# Autodesk Inventor assembly: Controlpanel
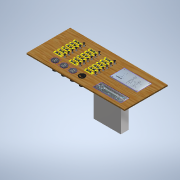
[picture p0: Inventor's stored thumbnail of the model, 180x180]
Saved by Autodesk Inventor 2021 (Build 250183000, 183)
## iProperties
Created: 2020-05-18
Part Number: Controlpanel
Document SubType Name: Assembly
Designer: Johansson
Author: Johansson
## Documents named in this file (10)
- C:\Users\oskar\Dropbox\Dokument\Projekt\Elita\Electrical system\Highside-Powerdistribution\hardware\control-panel\Controlpanel.iam
- C:\Users\oskar\Dropbox\Dokument\Projekt\Elita\Electrical system\Highside-Powerdistribution\hardware\control-panel\wooden-panel.ipt
- C:\Users\oskar\Dropbox\Dokument\Projekt\Elita\Electrical system\Highside-Powerdistribution\hardware\control-panel\label.ipt
- C:\Users\oskar\Dropbox\Dokument\Inventor\Content Center Files\R2019\en-US\CNS 9671\CNS 9671 - M2,3 x 5.ipt
- C:\Users\oskar\Dropbox\Dokument\Projekt\Elita\Electrical system\Highside-Powerdistribution\hardware\control-panel\stereo.ipt
- C:\Users\oskar\Dropbox\Dokument\Projekt\Elita\Electrical system\Highside-Powerdistribution\hardware\control-panel\usb_outlet.ipt
- C:\Users\oskar\Dropbox\Dokument\Projekt\Elita\Electrical system\Highside-Powerdistribution\hardware\control-panel\12v_outlet.ipt
- C:\Users\oskar\Dropbox\Dokument\Projekt\Elita\Electrical system\Highside-Powerdistribution\hardware\control-panel\dragswitch.ipt
- C:\Users\oskar\Dropbox\Dokument\Projekt\Elita\Electrical system\Highside-Powerdistribution\hardware\control-panel\infosign.ipt
- C:\Users\oskar\Dropbox\Dokument\Projekt\Elita\Electrical system\Highside-Powerdistribution\hardware\control-panel\parameters.xlsx
## Components (83 placed, 8 different names)
1. wooden-panel:1 — Mate:2, Mate:3, Mate:4, Mate:5, Mate:6, Mate:7, Mate:8, Mate:9, Mate:10, Mate:11, Mate:12
2. stereo:1 — Mate:3, Mate:4, Mate:5
3. 12v_outlet:1 — Mate:8, Mate:9
4. infosign:1 — Mate:12, Insert:5, Insert:6, Insert:7, Insert:8
5. CNS 9671 M2,3 x 5:45 — Insert:5
6. CNS 9671 M2,3 x 5:46 — Insert:6
7. CNS 9671 M2,3 x 5:47 — Insert:7
8. CNS 9671 M2,3 x 5:48 — Insert:8
9. label:5 — Mate:2, Insert:3, Insert:4
10. CNS 9671 M2,3 x 5:9 — Insert:3
11. CNS 9671 M2,3 x 5:10 — Insert:4
12. label:6
13. CNS 9671 M2,3 x 5:11
14. CNS 9671 M2,3 x 5:12
15. label:7
16. CNS 9671 M2,3 x 5:13
17. CNS 9671 M2,3 x 5:14
18. label:8
19. CNS 9671 M2,3 x 5:15
20. CNS 9671 M2,3 x 5:16
21. label:9
22. CNS 9671 M2,3 x 5:17
23. CNS 9671 M2,3 x 5:18
24. label:10
25. CNS 9671 M2,3 x 5:19
26. CNS 9671 M2,3 x 5:20
27. label:11
28. CNS 9671 M2,3 x 5:21
29. CNS 9671 M2,3 x 5:22
30. label:12
31. CNS 9671 M2,3 x 5:23
32. CNS 9671 M2,3 x 5:24
33. label:13
34. CNS 9671 M2,3 x 5:25
35. CNS 9671 M2,3 x 5:26
36. label:14
37. CNS 9671 M2,3 x 5:27
38. CNS 9671 M2,3 x 5:28
39. label:15
40. CNS 9671 M2,3 x 5:29
41. CNS 9671 M2,3 x 5:30
42. label:16
43. CNS 9671 M2,3 x 5:31
44. CNS 9671 M2,3 x 5:32
45. label:17
46. CNS 9671 M2,3 x 5:33
47. CNS 9671 M2,3 x 5:34
48. label:18
49. CNS 9671 M2,3 x 5:35
50. CNS 9671 M2,3 x 5:36
51. label:19
52. CNS 9671 M2,3 x 5:37
53. CNS 9671 M2,3 x 5:38
54. label:20
55. CNS 9671 M2,3 x 5:39
56. CNS 9671 M2,3 x 5:40
57. label:21
58. CNS 9671 M2,3 x 5:41
59. CNS 9671 M2,3 x 5:42
60. label:22
61. CNS 9671 M2,3 x 5:43
62. CNS 9671 M2,3 x 5:44
63. usb_outlet:1 — Mate:6, Mate:7
64. usb_outlet:2
65. usb_outlet:3
66. dragswitch:1 — Mate:10, Mate:11
67. dragswitch:2
68. dragswitch:3
69. dragswitch:4
70. dragswitch:5
71. dragswitch:6
72. dragswitch:7
73. dragswitch:8
74. dragswitch:9
75. dragswitch:10
76. dragswitch:11
77. dragswitch:12
78. dragswitch:13
79. dragswitch:14
80. dragswitch:15
81. dragswitch:16
82. dragswitch:17
83. dragswitch:18
## Component patterns: (18 elements, first: label:5 + CNS 9671 M2,3 x 5:9 + CNS 9671 M2,3 x 5:10), (3 elements, first: usb_outlet:1), (18 elements, first: dragswitch:1)
## Relationships (17: Mate 11, Insert 6)
- Mate:2: wooden-panel:1 ↔ label:5
- Insert:3: label:5 ↔ CNS 9671 M2,3 x 5:9
- Insert:4: label:5 ↔ CNS 9671 M2,3 x 5:10
- Mate:3: wooden-panel:1 ↔ stereo:1
- Mate:4: wooden-panel:1 ↔ stereo:1
- Mate:5: wooden-panel:1 ↔ stereo:1
- Mate:6: wooden-panel:1 ↔ usb_outlet:1
- Mate:7: wooden-panel:1 ↔ usb_outlet:1
- Mate:8: wooden-panel:1 ↔ 12v_outlet:1
- Mate:9: wooden-panel:1 ↔ 12v_outlet:1
- Mate:10: wooden-panel:1 ↔ dragswitch:1
- Mate:11: wooden-panel:1 ↔ dragswitch:1
- Mate:12: wooden-panel:1 ↔ infosign:1
- Insert:5: infosign:1 ↔ CNS 9671 M2,3 x 5:45
- Insert:6: infosign:1 ↔ CNS 9671 M2,3 x 5:46
- Insert:7: infosign:1 ↔ CNS 9671 M2,3 x 5:47
- Insert:8: infosign:1 ↔ CNS 9671 M2,3 x 5:48
## Named parameters: wl_panel = 285 mm, wr_panel = 280 mm, l_panel = 640 mm, t_panel = 8 mm, r_button = 8 mm, l_stereo = 178 mm, w_stereo = 50 mm, d_stereo = 177 mm, w_label = 15 mm, l_label = 50 mm, n_navlights = 4, r_labelscrew = 2.5 mm, ro_labelscrew = 5 mm, l_buttontobutton = 25 mm, n_interior = 6, r_usboutlet = 29 mm, n_usboutlets = 4, l_fastener_button = 19 mm, l_infosign = 180 mm, w_infosign = 100 mm
